# Autodesk Inventor assembly: bunny bot 2013 manipulator 2
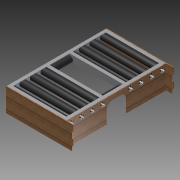
[picture p0: Inventor's stored thumbnail of the model, 180x180]
Saved by Autodesk Inventor 2012 (Build 160160000, 160)
## iProperties
Created: 2013-09-01
Part Number: bunny bot 2013 manipulator 2
Document SubType Name: Assembly
Designer: Bryce
Author: Bryce
## Documents named in this file (11)
- C:\Users\Bryce\Dropbox\Inventor Design Project Files\Independent Swerves\Inventor 2012\bunny bot 2013 manipulator 2.iam
- C:\Users\Bryce\Dropbox\Inventor Design Project Files\Independent Swerves\Inventor 2012\manipulator L frame right.ipt
- C:\Users\Bryce\Dropbox\Inventor Design Project Files\Independent Swerves\Inventor 2012\manipulator L frame left.ipt
- C:\Users\Bryce\Dropbox\Inventor Design Project Files\Independent Swerves\Inventor 2012\manipulator L frame middle.ipt
- C:\Users\Bryce\Dropbox\Inventor Design Project Files\Independent Swerves\Inventor 2012\manipulator centering shaft.ipt
- C:\Users\Bryce\Dropbox\Inventor Design Project Files\Independent Swerves\Inventor 2012\manipulator propeling shaft.ipt
- C:\Users\Bryce\Dropbox\Inventor Design Project Files\Independent Swerves\Inventor 2012\manipulator centering roller.ipt
- C:\Users\Bryce\Dropbox\Inventor Design Project Files\Independent Swerves\Inventor 2012\manipulator propeling roller.ipt
- C:\Users\Bryce\Dropbox\Inventor Design Project Files\Independent Swerves\Inventor 2012\maipulator L frame front 2.ipt
- C:\Users\Bryce\Dropbox\Inventor Design Project Files\Independent Swerves\Inventor 2012\manipulator back pannel 2.ipt
- C:\Users\Bryce\Dropbox\Inventor Design Project Files\Independent Swerves\Inventor 2012\manipulator side pannel 2.ipt
## Components (29 placed, 10 different names)
1. manipulator L frame right:1 — Mate:1, Mate:2, Flush:1, Mate:8, Mate:33, Flush:16
2. manipulator L frame left:1 — Mate:1, Mate:2, Flush:1, Mate:3, Flush:2, Flush:3, Mate:4, Flush:4, Flush:5, Mate:7, Mate:46, Flush:26
3. maipulator L frame front 2:1 — Mate:3, Flush:2, Flush:3, Mate:9, Mate:10, Mate:11, Mate:12, Flush:8, Flush:9, Flush:10, Flush:11, Mate:19, Mate:20, Mate:21, Mate:22, Mate:27, Mate:28, Flush:14, Flush:15, Mate:31, Mate:32, Flush:17, Mate:41, Flush:24, Mate:42, Mate:44, Mate:45, Flush:25, Flush:27
4. maipulator L frame front 2:2 — Mate:4, Flush:4, Flush:5, Mate:5, Mate:6, Flush:6, Flush:7, Flush:20, Mate:35
5. manipulator L frame middle:1 — Mate:6, Flush:6, Mate:7, Mate:25, Mate:26
6. manipulator L frame middle:2 — Mate:5, Flush:7, Mate:8, Mate:13, Flush:12, Mate:14, Flush:13
7. manipulator centering shaft:1 — Mate:10, Flush:9, Mate:16
8. manipulator centering shaft:2 — Mate:9, Flush:8, Mate:15
9. manipulator centering shaft:3 — Mate:11, Flush:10, Mate:17
10. manipulator centering shaft:4 — Mate:12, Flush:11, Mate:18
11. manipulator propeling shaft:1 — Mate:13, Flush:12, Mate:24
12. manipulator propeling shaft:2 — Mate:14, Flush:13, Mate:23
13. manipulator centering roller:1 — Mate:15, Mate:19
14. manipulator centering roller:2 — Mate:16, Mate:20
15. manipulator centering roller:3 — Mate:17, Mate:21
16. manipulator centering roller:4 — Mate:18, Mate:22
17. manipulator propeling roller:1 — Mate:24, Mate:26
18. manipulator propeling roller:2 — Mate:23, Mate:25
19. manipulator centering shaft:5 — Mate:27, Flush:14, Mate:29
20. manipulator centering shaft:6 — Mate:28, Flush:15, Mate:30
21. manipulator centering roller:5 — Mate:29, Mate:31
22. manipulator centering roller:6 — Mate:30, Mate:32
23. manipulator side pannel 2:1 — Mate:33, Flush:16, Flush:17, Mate:36
24. manipulator side pannel 2:2 — Mate:46, Flush:26, Flush:27
25. manipulator back pannel 2:1 — Flush:20, Mate:35, Mate:36
26. manipulator centering roller:7 — Mate:40, Mate:42
27. manipulator centering shaft:7 — Mate:40, Mate:41, Flush:24
28. manipulator centering roller:8 — Mate:43, Mate:45
29. manipulator centering shaft:8 — Mate:43, Mate:44, Flush:25
## Relationships (64: Mate 42, Flush 22)
- Mate:1: manipulator L frame right:1 ↔ manipulator L frame left:1
- Mate:2 (806.45 mm): manipulator L frame right:1 ↔ manipulator L frame left:1
- Flush:1: manipulator L frame right:1 ↔ manipulator L frame left:1
- Mate:3: manipulator L frame left:1 ↔ maipulator L frame front 2:1
- Flush:2: manipulator L frame left:1 ↔ maipulator L frame front 2:1
- Flush:3: manipulator L frame left:1 ↔ maipulator L frame front 2:1
- Mate:4: manipulator L frame left:1 ↔ maipulator L frame front 2:2
- Flush:4: manipulator L frame left:1 ↔ maipulator L frame front 2:2
- Flush:5: manipulator L frame left:1 ↔ maipulator L frame front 2:2
- Mate:5: maipulator L frame front 2:2 ↔ manipulator L frame middle:2
- Mate:6: maipulator L frame front 2:2 ↔ manipulator L frame middle:1
- Flush:6: maipulator L frame front 2:2 ↔ manipulator L frame middle:1
- Flush:7: maipulator L frame front 2:2 ↔ manipulator L frame middle:2
- Mate:7 (-323.85 mm): manipulator L frame left:1 ↔ manipulator L frame middle:1
- Mate:8 (-323.85 mm): manipulator L frame right:1 ↔ manipulator L frame middle:2
- Mate:9: maipulator L frame front 2:1 ↔ manipulator centering shaft:2
- Mate:10: maipulator L frame front 2:1 ↔ manipulator centering shaft:1
- Mate:11: maipulator L frame front 2:1 ↔ manipulator centering shaft:3
- Mate:12: maipulator L frame front 2:1 ↔ manipulator centering shaft:4
- Flush:8: maipulator L frame front 2:1 ↔ manipulator centering shaft:2
- Flush:9: maipulator L frame front 2:1 ↔ manipulator centering shaft:1
- Flush:10: maipulator L frame front 2:1 ↔ manipulator centering shaft:3
- Flush:11: maipulator L frame front 2:1 ↔ manipulator centering shaft:4
- Mate:13: manipulator L frame middle:2 ↔ manipulator propeling shaft:1
- Flush:12: manipulator L frame middle:2 ↔ manipulator propeling shaft:1
- Mate:14: manipulator L frame middle:2 ↔ manipulator propeling shaft:2
- Flush:13: manipulator L frame middle:2 ↔ manipulator propeling shaft:2
- Mate:15: manipulator centering shaft:2 ↔ manipulator centering roller:1
- Mate:16: manipulator centering shaft:1 ↔ manipulator centering roller:2
- Mate:17: manipulator centering shaft:3 ↔ manipulator centering roller:3
- Mate:18: manipulator centering shaft:4 ↔ manipulator centering roller:4
- Mate:19 (6.35 mm): maipulator L frame front 2:1 ↔ manipulator centering roller:1
- Mate:20 (6.35 mm): maipulator L frame front 2:1 ↔ manipulator centering roller:2
- Mate:21 (6.35 mm): maipulator L frame front 2:1 ↔ manipulator centering roller:3
- Mate:22 (6.35 mm): maipulator L frame front 2:1 ↔ manipulator centering roller:4
- Mate:23: manipulator propeling shaft:2 ↔ manipulator propeling roller:2
- Mate:24: manipulator propeling shaft:1 ↔ manipulator propeling roller:1
- Mate:25 (6.35 mm): manipulator L frame middle:1 ↔ manipulator propeling roller:2
- Mate:26 (6.35 mm): manipulator L frame middle:1 ↔ manipulator propeling roller:1
- Mate:27: maipulator L frame front 2:1 ↔ manipulator centering shaft:5
- Mate:28: maipulator L frame front 2:1 ↔ manipulator centering shaft:6
- Flush:14: maipulator L frame front 2:1 ↔ manipulator centering shaft:5
- Flush:15: maipulator L frame front 2:1 ↔ manipulator centering shaft:6
- Mate:29: manipulator centering shaft:5 ↔ manipulator centering roller:5
- Mate:30: manipulator centering shaft:6 ↔ manipulator centering roller:6
- Mate:31 (6.35 mm): maipulator L frame front 2:1 ↔ manipulator centering roller:5
- Mate:32 (6.35 mm): maipulator L frame front 2:1 ↔ manipulator centering roller:6
- Mate:33: manipulator L frame right:1 ↔ manipulator side pannel 2:1
- Flush:16: manipulator L frame right:1 ↔ manipulator side pannel 2:1
- Flush:17: maipulator L frame front 2:1 ↔ manipulator side pannel 2:1
- Flush:20: maipulator L frame front 2:2 ↔ manipulator back pannel 2:1
- Mate:35: maipulator L frame front 2:2 ↔ manipulator back pannel 2:1
- Mate:36: manipulator side pannel 2:1 ↔ manipulator back pannel 2:1
- Mate:40: manipulator centering roller:7 ↔ manipulator centering shaft:7
- Mate:41: maipulator L frame front 2:1 ↔ manipulator centering shaft:7
- Flush:24: maipulator L frame front 2:1 ↔ manipulator centering shaft:7
- Mate:42 (6.35 mm): maipulator L frame front 2:1 ↔ manipulator centering roller:7
- Mate:43: manipulator centering roller:8 ↔ manipulator centering shaft:8
- Mate:44: maipulator L frame front 2:1 ↔ manipulator centering shaft:8
- Mate:45 (6.35 mm): maipulator L frame front 2:1 ↔ manipulator centering roller:8
- Flush:25: maipulator L frame front 2:1 ↔ manipulator centering shaft:8
- Mate:46: manipulator L frame left:1 ↔ manipulator side pannel 2:2
- Flush:26: manipulator L frame left:1 ↔ manipulator side pannel 2:2
- Flush:27: maipulator L frame front 2:1 ↔ manipulator side pannel 2:2
